# Autodesk Inventor assembly: copyOfAmazonProductV01
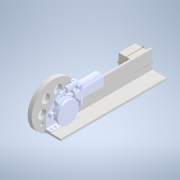
[picture p0: Inventor's stored thumbnail of the model, 180x180]
Saved by Autodesk Inventor 2020.2 (Build 242310000, 310)
## iProperties
Created: 2020-01-21
Part Number: copyOfAmazonProductV01
Document SubType Name: Assembly
Designer: robst
Author: robst
## Documents named in this file (9)
- C:\git\CAD-Development\robSteele\2020BallTriggerMechanism\copyOfAmazonProductV01.iam
- C:\git\CAD-Development\robSteele\2020BallTriggerMechanism\base.ipt
- C:\git\CAD-Development\robSteele\2020BallTriggerMechanism\am-2235a Snow Blower Motor With Hex Shaft.iam
- C:\git\CAD-Development\robSteele\2020BallTriggerMechanism\driveForPiston-4-in.ipt
- C:\git\CAD-Development\robSteele\2020BallTriggerMechanism\am-2373 Snow Blower Motor Mount.ipt
- C:\git\CAD-Development\robSteele\2020BallTriggerMechanism\connectingRod-4-in.ipt
- C:\git\CAD-Development\robSteele\2020BallTriggerMechanism\cylinderForCopy.ipt
- C:\git\CAD-Development\robSteele\2020BallTriggerMechanism\linearMotionRod.ipt
- C:\git\CAD-Development\robSteele\2020BallTriggerMechanism\tieRod.ipt
## Components (8 placed, 8 different names)
1. base:1 — Mate:1, Flush:1, Flush:2, Flush:3, Flush:4
2. am-2235a Snow Blower Motor With Hex Shaft:1 [sub-assembly] — Insert:1, Insert:2, Insert:3
3. driveForPiston-4-in:1 — Insert:3, Insert:4
4. am-2373 Snow Blower Motor Mount:1 — Mate:1, Flush:1, Flush:2, Insert:1, Insert:2
5. connectingRod-4-in:1 — Insert:4, Insert:5
6. cylinderForCopy:1 — Mate:2, Mate:3, Flush:3, Flush:4
7. linearMotionRod:1 — Insert:6, Mate:2, Mate:3
8. tieRod:1 — Insert:5, Insert:6
## Relationships (13: Insert 6, Flush 4, Mate 3)
- Mate:1: base:1 ↔ am-2373 Snow Blower Motor Mount:1
- Flush:1: base:1 ↔ am-2373 Snow Blower Motor Mount:1
- Flush:2: base:1 ↔ am-2373 Snow Blower Motor Mount:1
- Insert:1: am-2235a Snow Blower Motor With Hex Shaft:1 ↔ am-2373 Snow Blower Motor Mount:1
- Insert:2: am-2235a Snow Blower Motor With Hex Shaft:1 ↔ am-2373 Snow Blower Motor Mount:1
- Insert:3: am-2235a Snow Blower Motor With Hex Shaft:1 ↔ driveForPiston-4-in:1
- Insert:4: driveForPiston-4-in:1 ↔ connectingRod-4-in:1
- Insert:5: connectingRod-4-in:1 ↔ tieRod:1
- Insert:6 (-12.7 mm): linearMotionRod:1 ↔ tieRod:1
- Mate:2: cylinderForCopy:1 ↔ linearMotionRod:1
- Mate:3: cylinderForCopy:1 ↔ linearMotionRod:1
- Flush:3: base:1 ↔ cylinderForCopy:1
- Flush:4: base:1 ↔ cylinderForCopy:1
